# Autodesk Inventor assembly: Inner
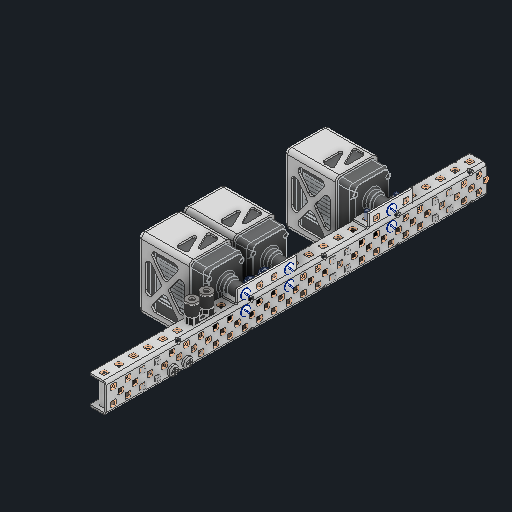
[picture p0: Inventor's stored thumbnail of the model, 512x512]
Saved by Autodesk Inventor 2025 (Build 290162000, 162)
## iProperties
Created: 2025-01-28
Part Number: Inner
Document SubType Name: Assembly
Designer: Averey Ku
Author: Averey Ku
## Documents named in this file (24)
- D:\VEX\High Stakes\CAD\V5\Chassis\Drivebay Left\Inner.iam
- D:\VEX\High Stakes\CAD\ROBOPROS-CAD-Inventor\Structure\C Channel\Aluminum 1x2x1\Alu C 1x2x1x26.ipt
- D:\VEX\High Stakes\CAD\ROBOPROS-CAD-Inventor\Electronics\Motor with Cover.iam
- D:\VEX\High Stakes\CAD\ROBOPROS-CAD-Inventor\Structure\C Channel\Aluminum 1x3x1 Half\Alu C Half 1x3x1x4.ipt
- D:\VEX\High Stakes\CAD\ROBOPROS-CAD-Inventor\Motion\Spacers\Spacer Nylon .313 OD\NSpacer .313 OD x .500.ipt
- D:\VEX\High Stakes\CAD\ROBOPROS-CAD-Inventor\Motion\Spacers\Spacer Nylon .313 OD.ipt
- D:\VEX\High Stakes\CAD\ROBOPROS-CAD-Inventor\Motion\Spacers\Washer Steel\SWasher .375 OD x .062500.ipt
- D:\VEX\High Stakes\CAD\ROBOPROS-CAD-Inventor\Motion\Spacers\Washer Steel.ipt
- D:\VEX\High Stakes\CAD\ROBOPROS-CAD-Inventor\Structure\Hardware\Screw Shoulder Robosource.ipt
- D:\VEX\High Stakes\CAD\ROBOPROS-CAD-Inventor\Structure\Hardware\Screw Shoulder Robosource\SScrew Shoulder Smooth .375 x .12.ipt
- D:\VEX\High Stakes\CAD\ROBOPROS-CAD-Inventor\Structure\Hardware\Nut Nylock.ipt
- D:\VEX\High Stakes\CAD\ROBOPROS-CAD-Inventor\Motion\Shaft LS\Bearing Flat Low Profile.ipt
- D:\VEX\High Stakes\CAD\ROBOPROS-CAD-Inventor\Structure\Hardware\Screw Nylon - Pan Head\NScrew Pan Head Threaded .500.ipt
- D:\VEX\High Stakes\CAD\ROBOPROS-CAD-Inventor\Structure\Hardware\Nut Nylon\Nut Nylon - White.ipt
- D:\VEX\High Stakes\CAD\ROBOPROS-CAD-Inventor\Structure\Hardware\Nut Nylon.ipt
- D:\VEX\High Stakes\CAD\ROBOPROS-CAD-Inventor\Structure\4-Post Hex Nut Retainer.ipt
- D:\VEX\High Stakes\CAD\ROBOPROS-CAD-Inventor\Structure\Nylon Standoff Rounded\Nylon Standoff .875.ipt
- D:\VEX\High Stakes\CAD\ROBOPROS-CAD-Inventor\Modified Parts\Bearing Flat Low Profile 2-Hole.ipt
- D:\VEX\High Stakes\CAD\ROBOPROS-CAD-Inventor\Motion\Spacers\Spacer Nylon .375 OD\NSpacer .375 OD x .375.ipt
- D:\VEX\High Stakes\CAD\ROBOPROS-CAD-Inventor\Motion\Spacers\Spacer Nylon .375 OD.ipt
- D:\VEX\High Stakes\CAD\ROBOPROS-CAD-Inventor\Structure\Standoff\Standoff .875.ipt
- D:\VEX\High Stakes\CAD\ROBOPROS-CAD-Inventor\Structure\Standoff.ipt
- D:\VEX\High Stakes\CAD\ROBOPROS-CAD-Inventor\Structure\Hardware\Screw Alu - Slotted\AScrew Slotted Threaded .250.ipt
- D:\VEX\High Stakes\CAD\ROBOPROS-CAD-Inventor\Structure\C Channel\Aluminum 1x3x1 Half\Alu C Half 1x3x1x3.ipt
## Components (40 placed, 17 different names)
1. Alu C 1x2x1x26:1 — Insert:10, Insert:31, Insert:34, Mate:8, Insert:37, Mate:9, Insert:39, Mate:10, Insert:40, Insert:41, Insert:42, Insert:49, Mate:11, Insert:50, Mate:12, Insert:52, Insert:53, Insert:58, Insert:59, Insert:60, Insert:61, Mate:14, Insert:65, Mate:15, Insert:70, Insert:72, Insert:73, Insert:75, Insert:76
2. Motor with Cover:1 [sub-assembly] — Insert:70, Mate:16
3. Motor with Cover:2 [sub-assembly] — Insert:71
4. Motor with Cover:3 [sub-assembly] — Insert:63, Mate:14
5. NSpacer .313 OD x .500:2 — Insert:10, Insert:12
6. SWasher .375 OD x .062500:1 — Insert:12
7. SScrew Shoulder Smooth .375 x .12:3 — Insert:59, Mate:13
8. Bearing Flat Low Profile:1 — Insert:50, Insert:51
9. NScrew Pan Head Threaded .500:1 — Insert:31
10. Nut Nylon - White:1 — Mate:12
11. Nut Nylon - White:2 — Insert:51
12. NScrew Pan Head Threaded .500:2 — Insert:52
13. 4-Post Hex Nut Retainer:1 — Insert:34, Mate:8, Insert:35
14. Nut Nylock:2 — Insert:35
15. 4-Post Hex Nut Retainer:2 — Insert:37, Mate:9
16. Nut Nylock:3
17. 4-Post Hex Nut Retainer:3 — Insert:39, Mate:10
18. Nut Nylock:4
19. Nylon Standoff .875:1 — Insert:40
20. Nut Nylock:5 — Insert:66
21. Nut Nylock:6 — Insert:67
22. SScrew Shoulder Smooth .375 x .12:4 — Insert:41
23. SScrew Shoulder Smooth .375 x .12:5 — Insert:42
24. Bearing Flat Low Profile 2-Hole:1 — Insert:49
25. NSpacer .375 OD x .375:1
26. SWasher .375 OD x .062500:4 — Mate:11
27. NSpacer .375 OD x .375:2
28. SWasher .375 OD x .062500:5
29. Standoff .875:1 — Insert:53
30. AScrew Slotted Threaded .250:1 — Insert:68
31. AScrew Slotted Threaded .250:2 — Insert:69
32. AScrew Slotted Threaded .250:3 — Insert:58
33. SScrew Shoulder Smooth .375 x .12:6 — Insert:60
34. Alu C Half 1x3x1x3:1 — Insert:61, Mate:13, Insert:63, Insert:74
35. Alu C Half 1x3x1x4:2 — Insert:65, Mate:15, Insert:66, Insert:67, Insert:68, Insert:69, Mate:16, Insert:71
36. AScrew Slotted Threaded .250:4 — Insert:73
37. AScrew Slotted Threaded .250:5 — Insert:72
38. AScrew Slotted Threaded .250:6 — Insert:75
39. AScrew Slotted Threaded .250:7 — Insert:74
40. Nylon Standoff .875:2 — Insert:76
## Relationships (51: Insert 39, Mate 12)
- [Mate]: Alu C 1x2x1x26:1 ↔ Motor with Cover:1
- [Mate]: Alu C 1x2x1x26:1 ↔ Motor with Cover:2
- [Mate]: Alu C 1x2x1x26:1 ↔ Motor with Cover:3
- Insert:10: Alu C 1x2x1x26:1 ↔ NSpacer .313 OD x .500:2
- Insert:12: NSpacer .313 OD x .500:2 ↔ SWasher .375 OD x .062500:1
- [Insert] (1.27 mm): Bearing Flat Low Profile:1 ↔ Nut Nylon - White:1
- Insert:31: Alu C 1x2x1x26:1 ↔ NScrew Pan Head Threaded .500:1
- Insert:34: Alu C 1x2x1x26:1 ↔ 4-Post Hex Nut Retainer:1
- Mate:8: Alu C 1x2x1x26:1 ↔ 4-Post Hex Nut Retainer:1
- Insert:35: 4-Post Hex Nut Retainer:1 ↔ Nut Nylock:2
- [Insert]: 4-Post Hex Nut Retainer:2 ↔ Nut Nylock:3
- Insert:37: Alu C 1x2x1x26:1 ↔ 4-Post Hex Nut Retainer:2
- Mate:9: Alu C 1x2x1x26:1 ↔ 4-Post Hex Nut Retainer:2
- [Insert]: 4-Post Hex Nut Retainer:3 ↔ Nut Nylock:4
- Insert:39: Alu C 1x2x1x26:1 ↔ 4-Post Hex Nut Retainer:3
- Mate:10: Alu C 1x2x1x26:1 ↔ 4-Post Hex Nut Retainer:3
- Insert:40: Alu C 1x2x1x26:1 ↔ Nylon Standoff .875:1
- Insert:41: Alu C 1x2x1x26:1 ↔ SScrew Shoulder Smooth .375 x .12:4
- Insert:42: Alu C 1x2x1x26:1 ↔ SScrew Shoulder Smooth .375 x .12:5
- [Insert]: NSpacer .375 OD x .375:1 ↔ SWasher .375 OD x .062500:4
- [Insert] (1.27 mm): Bearing Flat Low Profile 2-Hole:1 ↔ NSpacer .375 OD x .375:1
- [Insert]: NSpacer .375 OD x .375:2 ↔ SWasher .375 OD x .062500:5
- [Insert] (1.27 mm): Bearing Flat Low Profile 2-Hole:1 ↔ NSpacer .375 OD x .375:2
- Insert:49: Alu C 1x2x1x26:1 ↔ Bearing Flat Low Profile 2-Hole:1
- Mate:11: Alu C 1x2x1x26:1 ↔ SWasher .375 OD x .062500:4
- Insert:50: Alu C 1x2x1x26:1 ↔ Bearing Flat Low Profile:1
- Mate:12: Alu C 1x2x1x26:1 ↔ Nut Nylon - White:1
- Insert:51 (1.27 mm): Bearing Flat Low Profile:1 ↔ Nut Nylon - White:2
- Insert:52: Alu C 1x2x1x26:1 ↔ NScrew Pan Head Threaded .500:2
- Insert:53: Alu C 1x2x1x26:1 ↔ Standoff .875:1
- Insert:58: Alu C 1x2x1x26:1 ↔ AScrew Slotted Threaded .250:3
- Insert:59: Alu C 1x2x1x26:1 ↔ SScrew Shoulder Smooth .375 x .12:3
- Insert:60: Alu C 1x2x1x26:1 ↔ SScrew Shoulder Smooth .375 x .12:6
- Insert:61: Alu C 1x2x1x26:1 ↔ Alu C Half 1x3x1x3:1
- Mate:13: SScrew Shoulder Smooth .375 x .12:3 ↔ Alu C Half 1x3x1x3:1
- Insert:63: Motor with Cover:3 ↔ Alu C Half 1x3x1x3:1
- Mate:14: Alu C 1x2x1x26:1 ↔ Motor with Cover:3
- Insert:65: Alu C 1x2x1x26:1 ↔ Alu C Half 1x3x1x4:2
- Mate:15: Alu C 1x2x1x26:1 ↔ Alu C Half 1x3x1x4:2
- Insert:66: Nut Nylock:5 ↔ Alu C Half 1x3x1x4:2
- Insert:67: Nut Nylock:6 ↔ Alu C Half 1x3x1x4:2
- Insert:68: AScrew Slotted Threaded .250:1 ↔ Alu C Half 1x3x1x4:2
- Insert:69: AScrew Slotted Threaded .250:2 ↔ Alu C Half 1x3x1x4:2
- Insert:70: Alu C 1x2x1x26:1 ↔ Motor with Cover:1
- Mate:16: Motor with Cover:1 ↔ Alu C Half 1x3x1x4:2
- Insert:71: Motor with Cover:2 ↔ Alu C Half 1x3x1x4:2
- Insert:72: Alu C 1x2x1x26:1 ↔ AScrew Slotted Threaded .250:5
- Insert:73: Alu C 1x2x1x26:1 ↔ AScrew Slotted Threaded .250:4
- Insert:74: Alu C Half 1x3x1x3:1 ↔ AScrew Slotted Threaded .250:7
- Insert:75: Alu C 1x2x1x26:1 ↔ AScrew Slotted Threaded .250:6
- Insert:76: Alu C 1x2x1x26:1 ↔ Nylon Standoff .875:2
## Named parameters: d52_d51 = 0 mm, d55_d51 = 0 mm, d102_d100 = 0 mm
